# Autodesk Inventor assembly: FULL
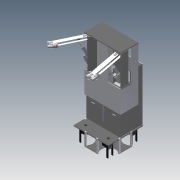
[picture p0: Inventor's stored thumbnail of the model, 180x180]
Saved by Autodesk Inventor 2011 (Build 150239000, 239)
## iProperties
Created: 2011-09-17
Part Number: FULL
Document SubType Name: Assembly
Designer: Matthew
Author: Matthew
## Documents named in this file (10)
- C:\Users\Matthew\Documents\matthew_autocad\prlite\FULL.iam
- C:\Users\Matthew\Documents\matthew_autocad\prlite\base\BASE.iam
- C:\Users\Matthew\Documents\matthew_autocad\prlite\inner torso\INNER TORSO.iam
- C:\Users\Matthew\Documents\matthew_autocad\prlite\slider\1.ipt
- C:\Users\Matthew\Documents\matthew_autocad\prlite\slider\2.ipt
- C:\Users\Matthew\Documents\matthew_autocad\prlite\outer torso\OUTER TORSO.iam
- C:\Users\Matthew\Documents\matthew_autocad\prlite\lazy susan\1.ipt
- C:\Users\Matthew\Documents\matthew_autocad\prlite\lazy susan\2.ipt
- C:\Users\Matthew\Documents\matthew_autocad\prlite\wheel\wheelholder2.iam
- C:\Users\Matthew\Documents\matthew_autocad\prlite\wheel\wheelholder1.iam
## Components (17 placed, 7 different names)
1. BASE:1 [sub-assembly] — Mate:25, Mate:26, Mate:27, Mate:28, Mate:29, Mate:30, Mate:31, Mate:32, Mate:33, Mate:34, Mate:35, Mate:36, Mate:41, Flush:4, Flush:5
2. INNER TORSO:1 [sub-assembly] — Mate:8, Mate:15, Mate:16, Mate:40, Mate:41, Flush:4, Flush:5
3. 1:2 — Mate:8, Mate:13, Mate:14, Flush:2, Mate:15, Mate:16, Mate:40
4. 2:1 — Mate:13, Mate:14, Flush:2, Mate:37, Mate:38, Mate:39
5. 1:3 — Mate:23, Mate:24, Mate:48, Mate:49, Mate:50
6. 1:4 — Mate:21, Mate:22, Mate:45, Mate:46, Mate:47
7. 1:5 — Mate:19, Mate:20, Mate:51, Mate:52, Mate:53
8. 1:6 — Mate:17, Mate:18, Mate:42, Mate:43, Mate:44
9. 2:2 — Mate:17, Mate:18, Mate:30, Mate:31, Mate:32
10. 2:3 — Mate:21, Mate:22, Mate:28, Mate:33, Mate:34
11. 2:4 — Mate:19, Mate:20, Mate:29, Mate:35, Mate:36
12. 2:5 — Mate:23, Mate:24, Mate:25, Mate:26, Mate:27
13. OUTER TORSO:1 [sub-assembly] — Mate:37, Mate:38, Mate:39
14. wheelholder2:1 [sub-assembly] — Mate:45, Mate:46, Mate:47
15. wheelholder2:2 [sub-assembly] — Mate:42, Mate:43, Mate:44
16. wheelholder1:1 [sub-assembly] — Mate:48, Mate:49, Mate:50
17. wheelholder1:2 [sub-assembly] — Mate:51, Mate:52, Mate:53
## Relationships (45: Mate 42, Flush 3)
- Mate:8: INNER TORSO:1 ↔ 1:2
- Mate:13: 1:2 ↔ 2:1
- Mate:14: 1:2 ↔ 2:1
- Flush:2: 1:2 ↔ 2:1
- Mate:15: INNER TORSO:1 ↔ 1:2
- Mate:16: INNER TORSO:1 ↔ 1:2
- Mate:17: 1:6 ↔ 2:2
- Mate:18: 1:6 ↔ 2:2
- Mate:19: 1:5 ↔ 2:4
- Mate:20: 1:5 ↔ 2:4
- Mate:21: 1:4 ↔ 2:3
- Mate:22: 1:4 ↔ 2:3
- Mate:23: 1:3 ↔ 2:5
- Mate:24: 1:3 ↔ 2:5
- Mate:25: BASE:1 ↔ 2:5
- Mate:26: BASE:1 ↔ 2:5
- Mate:27: BASE:1 ↔ 2:5
- Mate:28: BASE:1 ↔ 2:3
- Mate:29: BASE:1 ↔ 2:4
- Mate:30: BASE:1 ↔ 2:2
- Mate:31: BASE:1 ↔ 2:2
- Mate:32: BASE:1 ↔ 2:2
- Mate:33: BASE:1 ↔ 2:3
- Mate:34: BASE:1 ↔ 2:3
- Mate:35: BASE:1 ↔ 2:4
- Mate:36: BASE:1 ↔ 2:4
- Mate:37: 2:1 ↔ OUTER TORSO:1
- Mate:38: 2:1 ↔ OUTER TORSO:1
- Mate:39: 2:1 ↔ OUTER TORSO:1
- Mate:40: INNER TORSO:1 ↔ 1:2
- Mate:41: BASE:1 ↔ INNER TORSO:1
- Flush:4: BASE:1 ↔ INNER TORSO:1
- Flush:5 (6.35 mm): BASE:1 ↔ INNER TORSO:1
- Mate:42: 1:6 ↔ wheelholder2:2
- Mate:43: 1:6 ↔ wheelholder2:2
- Mate:44: 1:6 ↔ wheelholder2:2
- Mate:45: 1:4 ↔ wheelholder2:1
- Mate:46: 1:4 ↔ wheelholder2:1
- Mate:47: 1:4 ↔ wheelholder2:1
- Mate:48: 1:3 ↔ wheelholder1:1
- Mate:49: 1:3 ↔ wheelholder1:1
- Mate:50: 1:3 ↔ wheelholder1:1
- Mate:51: 1:5 ↔ wheelholder1:2
- Mate:52: 1:5 ↔ wheelholder1:2
- Mate:53: 1:5 ↔ wheelholder1:2
